# Autodesk Inventor assembly: Digitalmodul Baugruppe
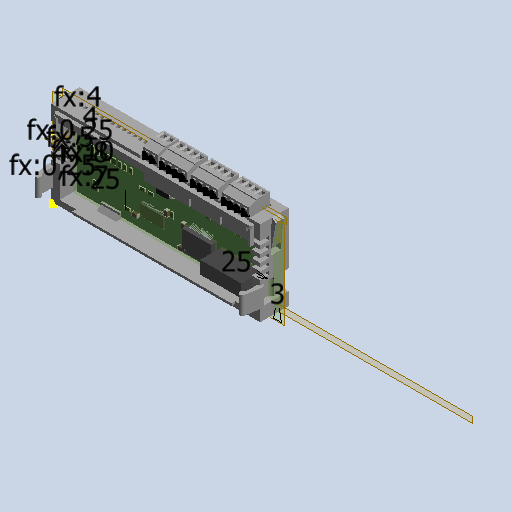
[picture p0: Inventor's stored thumbnail of the model, 512x512]
Saved by Autodesk Inventor 2025.2 (Build 292293000, 293)
## iProperties
Part Number: Digitalmodul Baugruppe
Document SubType Name: Baugruppe
Designer: leowa
Author: leowa
## Documents named in this file (6)
- C:\Users\leowa\OneDrive - Fachhochschule Aachen\FH\8. Semester\CAN Tram CAD\Module\Digitalmodul Baugruppe.iam
- C:\Users\leowa\OneDrive - Fachhochschule Aachen\FH\8. Semester\CAN Tram CAD\Gehäuse\Generisches Gehäuse V2.ipt
- C:\Users\leowa\OneDrive - Fachhochschule Aachen\FH\8. Semester\CAN Tram CAD\Platinen\Digitalmodul\Digitalmodul\Digitalmodul.iam
- C:\Users\leowa\OneDrive - Fachhochschule Aachen\FH\8. Semester\CAN Tram CAD\Gehäuse\Digitalmodul Gehäuse Deckel.ipt
- C:\Users\leowa\OneDrive - Fachhochschule Aachen\FH\8. Semester\CAN Tram CAD\Kaufteile\Terminalstecker 4fach\0395000004.iam
- C:\Users\leowa\OneDrive - Fachhochschule Aachen\FH\8. Semester\CAN Tram CAD\Kaufteile\Terminalstecker 2fach\0395000002.iam
## Components (7 placed, 5 different names)
1. Generisches Gehäuse V2:1 — Passend:1, Passend:2, Passend:3, Fluchtend:1, Fluchtend:2, Passend:4
2. Digitalmodul:1 [sub-assembly] — Passend:1, Passend:2, Passend:3, Passend:5, Passend:6, Passend:7, Passend:8, Passend:9, Passend:10, Passend:11, Passend:12, Passend:13, Passend:14, Passend:15, Passend:16
3. Digitalmodul Gehäuse Deckel:1 — Fluchtend:1, Fluchtend:2, Passend:4
4. 0395000004:1 [sub-assembly] — Passend:5, Passend:10, Passend:11
5. 0395000004:2 [sub-assembly] — Passend:6, Passend:9, Passend:12
6. 0395000004:3 [sub-assembly] — Passend:7, Passend:8, Passend:13
7. 0395000002:1 [sub-assembly] — Passend:14, Passend:15, Passend:16
## Relationships (18: Mate 16, Flush 2)
- Passend:1 [Mate]: Generisches Gehäuse V2:1 ↔ Digitalmodul:1
- Passend:2 [Mate]: Generisches Gehäuse V2:1 ↔ Digitalmodul:1
- Passend:3 [Mate] (1 mm): Generisches Gehäuse V2:1 ↔ Digitalmodul:1
- Fluchtend:1 [Flush]: Generisches Gehäuse V2:1 ↔ Digitalmodul Gehäuse Deckel:1
- Fluchtend:2 [Flush]: Generisches Gehäuse V2:1 ↔ Digitalmodul Gehäuse Deckel:1
- Passend:4 [Mate]: Generisches Gehäuse V2:1 ↔ Digitalmodul Gehäuse Deckel:1
- Passend:5 [Mate]: Digitalmodul:1 ↔ 0395000004:1
- Passend:6 [Mate]: Digitalmodul:1 ↔ 0395000004:2
- Passend:7 [Mate]: Digitalmodul:1 ↔ 0395000004:3
- Passend:8 [Mate]: Digitalmodul:1 ↔ 0395000004:3
- Passend:9 [Mate]: Digitalmodul:1 ↔ 0395000004:2
- Passend:10 [Mate]: Digitalmodul:1 ↔ 0395000004:1
- Passend:11 [Mate]: Digitalmodul:1 ↔ 0395000004:1
- Passend:12 [Mate]: Digitalmodul:1 ↔ 0395000004:2
- Passend:13 [Mate]: Digitalmodul:1 ↔ 0395000004:3
- Passend:14 [Mate]: Digitalmodul:1 ↔ 0395000002:1
- Passend:15 [Mate]: Digitalmodul:1 ↔ 0395000002:1
- Passend:16 [Mate]: Digitalmodul:1 ↔ 0395000002:1
